# Autodesk Inventor assembly: BV-ASM-222-104
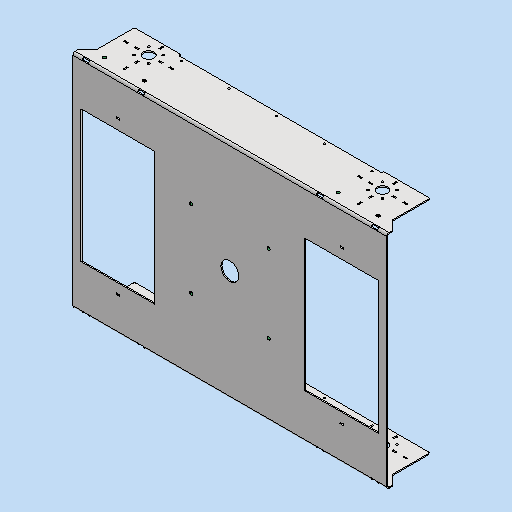
[picture p0: Inventor's stored thumbnail of the model, 512x512]
Saved by Autodesk Inventor 2025.3 (Build 293356030, 356C)
## iProperties
Created: 2025-12-10
Part Number: BV-ASM-222-104
Document SubType Name: Assembly
Designer: josh
Mass: 49946.6 g
Surface Area: 27394.5 cm^2
Volume: 6362.62 cm^3
Density: 7.85 g/cm^3
Description: BASE WELDMENT TOP HALF
Author: josh
## Documents named in this file (3)
- R:\A1- Neuweg Design Data\OM Robotics\BASE VEHICLE DESIGN PROJECT\BV-ASM-222-104.iam
- R:\A1- Neuweg Design Data\OM Robotics\BASE VEHICLE DESIGN PROJECT\BV-222-101.ipt
- R:\A1- Neuweg Design Data\OM Robotics\BASE VEHICLE DESIGN PROJECT\93560A112.ipt
## Components (13 placed, 2 different names)
1. BV-222-101:1 — Insert:1
2. 93560A112:2
3. 93560A112:3
4. 93560A112:4
5. 93560A112:5
6. 93560A112:6
7. 93560A112:7
8. 93560A112:8
9. 93560A112:9
10. 93560A112:1
11. 93560A112:10
12. 93560A112:11
13. 93560A112:12 — Insert:1
## Relationships (1: Insert 1)
- Insert:1: BV-222-101:1 ↔ 93560A112:12
